# Autodesk Inventor assembly: Telaio - Taglio
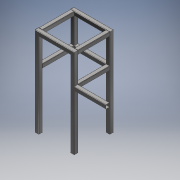
[picture p0: Inventor's stored thumbnail of the model, 180x180]
Saved by Autodesk Inventor 2018 (Build 220112000, 112)
## iProperties
Created: 2020-06-01
Part Number: Telaio - Taglio
Material: Generico
Document SubType Name: Assembly
Designer: Francesco
Author: Francesco
## Documents named in this file (4)
- C:\Users\Francesco\no-brim\Meccanica\Progetto Inventor no-brim\Assiemi\Telaio - Taglio.iam
- C:\Users\Francesco\no-brim\Meccanica\Progetto Inventor no-brim\Parti\Tubolare verticale 45 - Taglio.ipt
- C:\Users\Francesco\no-brim\Meccanica\Progetto Inventor no-brim\Parti\Tubolare horizontal 45 - Taglio.ipt
- C:\Users\Francesco\no-brim\Meccanica\Progetto Inventor no-brim\Parti\Tubolare horizontal - Taglio.ipt
## Components (12 placed, 3 different names)
1. Tubolare verticale 45 - Taglio:1 — Coincidente:1, Allineato:1, Coincidente:2, Allineato:3, Coincidente:11, Allineato:10
2. Tubolare verticale 45 - Taglio:2 — Allineato:3, Coincidente:5, Allineato:4, Coincidente:6, Coincidente:12, Allineato:11, Allineato:12
3. Tubolare verticale 45 - Taglio:3 — Coincidente:7, Allineato:5, Coincidente:8, Allineato:8, Coincidente:13, Coincidente:14, Allineato:14
4. Tubolare verticale 45 - Taglio:4 — Coincidente:3, Allineato:2, Coincidente:4, Coincidente:10, Coincidente:16, Allineato:17
5. Tubolare horizontal 45 - Taglio:1 — Coincidente:1, Allineato:1, Coincidente:2, Coincidente:3, Allineato:2, Coincidente:4, Allineato:6, Allineato:7
6. Tubolare horizontal 45 - Taglio:2 — Coincidente:5, Allineato:4, Coincidente:6, Coincidente:7, Allineato:5, Coincidente:8, Allineato:6, Coincidente:9
7. Tubolare horizontal - Taglio:1 — Coincidente:9, Allineato:7, Allineato:8, Coincidente:10, Allineato:9
8. Tubolare horizontal - Taglio:2 — Coincidente:11, Allineato:9, Allineato:10, Coincidente:15
9. Tubolare horizontal - Taglio:3 — Coincidente:14, Allineato:14, Allineato:15, Allineato:16
10. Tubolare horizontal - Taglio:4 — Coincidente:13, Allineato:12, Allineato:13, Allineato:15
11. Tubolare horizontal - Taglio:5 — Coincidente:12, Allineato:11, Allineato:13, Coincidente:15
12. Tubolare horizontal - Taglio:6 — Coincidente:16, Allineato:16, Allineato:17
## Relationships (33: Flush 17, Mate 16)
- Coincidente:1 [Mate]: Tubolare verticale 45 - Taglio:1 ↔ Tubolare horizontal 45 - Taglio:1
- Allineato:1 [Flush]: Tubolare verticale 45 - Taglio:1 ↔ Tubolare horizontal 45 - Taglio:1
- Coincidente:2 [Mate]: Tubolare verticale 45 - Taglio:1 ↔ Tubolare horizontal 45 - Taglio:1
- Coincidente:3 [Mate]: Tubolare verticale 45 - Taglio:4 ↔ Tubolare horizontal 45 - Taglio:1
- Allineato:2 [Flush]: Tubolare verticale 45 - Taglio:4 ↔ Tubolare horizontal 45 - Taglio:1
- Coincidente:4 [Mate]: Tubolare verticale 45 - Taglio:4 ↔ Tubolare horizontal 45 - Taglio:1
- Allineato:3 [Flush]: Tubolare verticale 45 - Taglio:1 ↔ Tubolare verticale 45 - Taglio:2
- Coincidente:5 [Mate]: Tubolare verticale 45 - Taglio:2 ↔ Tubolare horizontal 45 - Taglio:2
- Allineato:4 [Flush]: Tubolare verticale 45 - Taglio:2 ↔ Tubolare horizontal 45 - Taglio:2
- Coincidente:6 [Mate]: Tubolare verticale 45 - Taglio:2 ↔ Tubolare horizontal 45 - Taglio:2
- Coincidente:7 [Mate]: Tubolare verticale 45 - Taglio:3 ↔ Tubolare horizontal 45 - Taglio:2
- Allineato:5 [Flush]: Tubolare verticale 45 - Taglio:3 ↔ Tubolare horizontal 45 - Taglio:2
- Coincidente:8 [Mate]: Tubolare verticale 45 - Taglio:3 ↔ Tubolare horizontal 45 - Taglio:2
- Allineato:6 [Flush]: Tubolare horizontal 45 - Taglio:1 ↔ Tubolare horizontal 45 - Taglio:2
- Coincidente:9 [Mate]: Tubolare horizontal 45 - Taglio:2 ↔ Tubolare horizontal - Taglio:1
- Allineato:7 [Flush]: Tubolare horizontal 45 - Taglio:1 ↔ Tubolare horizontal - Taglio:1
- Allineato:8 [Flush]: Tubolare verticale 45 - Taglio:3 ↔ Tubolare horizontal - Taglio:1
- Coincidente:10 [Mate]: Tubolare verticale 45 - Taglio:4 ↔ Tubolare horizontal - Taglio:1
- Coincidente:11 [Mate]: Tubolare verticale 45 - Taglio:1 ↔ Tubolare horizontal - Taglio:2
- Allineato:9 [Flush]: Tubolare horizontal - Taglio:1 ↔ Tubolare horizontal - Taglio:2
- Allineato:10 [Flush]: Tubolare verticale 45 - Taglio:1 ↔ Tubolare horizontal - Taglio:2
- Coincidente:12 [Mate]: Tubolare verticale 45 - Taglio:2 ↔ Tubolare horizontal - Taglio:5
- Allineato:11 [Flush]: Tubolare verticale 45 - Taglio:2 ↔ Tubolare horizontal - Taglio:5
- Coincidente:13 [Mate]: Tubolare verticale 45 - Taglio:3 ↔ Tubolare horizontal - Taglio:4
- Allineato:12 [Flush]: Tubolare verticale 45 - Taglio:2 ↔ Tubolare horizontal - Taglio:4
- Allineato:13 [Flush]: Tubolare horizontal - Taglio:4 ↔ Tubolare horizontal - Taglio:5
- Coincidente:14 [Mate]: Tubolare verticale 45 - Taglio:3 ↔ Tubolare horizontal - Taglio:3
- Allineato:14 [Flush]: Tubolare verticale 45 - Taglio:3 ↔ Tubolare horizontal - Taglio:3
- Allineato:15 [Flush]: Tubolare horizontal - Taglio:3 ↔ Tubolare horizontal - Taglio:4
- Coincidente:15 [Mate] (260 mm): Tubolare horizontal - Taglio:2 ↔ Tubolare horizontal - Taglio:5
- Coincidente:16 [Mate]: Tubolare verticale 45 - Taglio:4 ↔ Tubolare horizontal - Taglio:6
- Allineato:16 [Flush]: Tubolare horizontal - Taglio:3 ↔ Tubolare horizontal - Taglio:6
- Allineato:17 [Flush]: Tubolare verticale 45 - Taglio:4 ↔ Tubolare horizontal - Taglio:6
